# Autodesk Inventor assembly: WheelAssembly
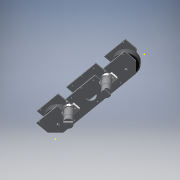
[picture p0: Inventor's stored thumbnail of the model, 180x180]
Saved by Autodesk Inventor 2017 (Build 210142000, 142)
## iProperties
Created: 2016-09-10
Part Number: WheelAssembly
Document SubType Name: Assembly
Designer: RoboticsUser
Author: RoboticsUser
## Documents named in this file (11)
- C:\Robotics\CAD\2016-17_CAD\WheelAssemblyRight.iam
- C:\Robotics\CAD\2015-16_CAD\custom cad parts\am-2648_4inWheel8mmHub.ipt
- C:\Robotics\CAD\COTSParts\Actobotics\545 parts\545556.ipt
- C:\Robotics\CAD\COTSParts\Actobotics\615 parts\615102.ipt
- C:\Robotics\CAD\COTSParts\Actobotics\634 parts\634080.ipt
- C:\Robotics\CAD\COTSParts\Motors\Andymark 2964  NeveRest 40 Motor.ipt
- C:\Users\RoboticsUser\Desktop\2015-16 CAD\COTSParts\Actobotics\615 parts\615114.ipt
- C:\Robotics\CAD\COTSParts\Tetrix\tetrix-motor-mounts-1.snapshot.1\Tetrex 2pc motor mount.ipt
- C:\Robotics\CAD\2016-17_CAD\DriveTrainPlateInside1.iam
- C:\Robotics\CAD\COTSParts\Actobotics\545 parts\545456.ipt
- C:\Robotics\CAD\2016-17_CAD\DriveTrainPlateOutside2.iam
## Components (22 placed, 10 different names)
1. am-2648_4inWheel8mmHub:2 — Insert:71, Insert:77
2. 545556:2 — Insert:72
3. 615102:4 — Insert:44, Insert:77
4. 634080:2 — Insert:70, Insert:78
5. am-2648_4inWheel8mmHub:3 — Insert:73, Insert:74
6. 545556:6 — Insert:75
7. 615102:5 — Insert:54
8. 634080:3 — Insert:66, Insert:79
9. Andymark 2964  NeveRest 40 Motor:2 — Insert:27, Insert:60
10. 545556:8 — Insert:61
11. 615114:2 — Insert:60, Insert:61
12. 615114:3 — Insert:58, Insert:59
13. 545556:9 — Insert:59
14. Andymark 2964  NeveRest 40 Motor:3 — Insert:28, Insert:58
15. Tetrex 2pc motor mount:1 — Insert:27, Insert:62, Insert:63
16. Tetrex 2pc motor mount:2 — Insert:28, Insert:64, Insert:65
17. DriveTrainPlateInside1:1 [sub-assembly] — Insert:62, Insert:63, Insert:64, Insert:65, Insert:66, Insert:67, Insert:70, Insert:76
18. 545556:10 — Insert:44, Insert:76
19. 545456:1 — Insert:71, Insert:72
20. 545456:3 — Insert:74, Insert:75
21. 545556:11 — Insert:54, Insert:67, Insert:73
22. DriveTrainPlateOutside2:1 [sub-assembly] — Insert:78, Insert:79
## Relationships (24: Insert 24)
- Insert:27 (6.35 mm): Andymark 2964  NeveRest 40 Motor:2 ↔ Tetrex 2pc motor mount:1
- Insert:28 (6.35 mm): Andymark 2964  NeveRest 40 Motor:3 ↔ Tetrex 2pc motor mount:2
- Insert:44: 615102:4 ↔ 545556:10
- Insert:54: 615102:5 ↔ 545556:11
- Insert:58 (16.0274 mm): 615114:3 ↔ Andymark 2964  NeveRest 40 Motor:3
- Insert:59: 615114:3 ↔ 545556:9
- Insert:60 (16.0274 mm): Andymark 2964  NeveRest 40 Motor:2 ↔ 615114:2
- Insert:61: 545556:8 ↔ 615114:2
- Insert:62: Tetrex 2pc motor mount:1 ↔ DriveTrainPlateInside1:1
- Insert:63: Tetrex 2pc motor mount:1 ↔ DriveTrainPlateInside1:1
- Insert:64: Tetrex 2pc motor mount:2 ↔ DriveTrainPlateInside1:1
- Insert:65: Tetrex 2pc motor mount:2 ↔ DriveTrainPlateInside1:1
- Insert:66 (-6.35 mm): 634080:3 ↔ DriveTrainPlateInside1:1
- Insert:67 (3.175 mm): DriveTrainPlateInside1:1 ↔ 545556:11
- Insert:70 (-6.35 mm): 634080:2 ↔ DriveTrainPlateInside1:1
- Insert:71: am-2648_4inWheel8mmHub:2 ↔ 545456:1
- Insert:72: 545556:2 ↔ 545456:1
- Insert:73 (9.525 mm): am-2648_4inWheel8mmHub:3 ↔ 545556:11
- Insert:74: am-2648_4inWheel8mmHub:3 ↔ 545456:3
- Insert:75: 545556:6 ↔ 545456:3
- Insert:76 (3.175 mm): DriveTrainPlateInside1:1 ↔ 545556:10
- Insert:77 (9.525 mm): am-2648_4inWheel8mmHub:2 ↔ 615102:4
- Insert:78 (19.05 mm): 634080:2 ↔ DriveTrainPlateOutside2:1
- Insert:79 (19.05 mm): 634080:3 ↔ DriveTrainPlateOutside2:1
